# Autodesk Inventor assembly: Power Supply Board
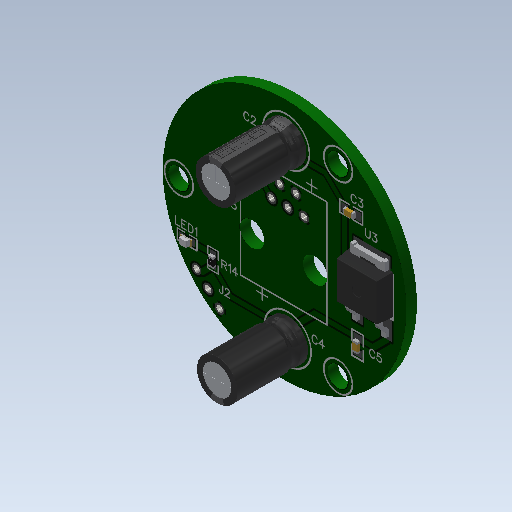
[picture p0: Inventor's stored thumbnail of the model, 512x512]
Saved by Autodesk Inventor 2020 (Build 240168000, 168)
## iProperties
Created: 2018-05-01
Part Number: Power Supply Board
Document SubType Name: Assembly
Designer: Alex
Description: 5V Regulator with RJ12 Interface
Author: Alex
## Documents named in this file (7)
- C:\Users\amsmi\Google Drive\Pirani Gauge\Pirani Gauge Modeling\Gauge Rev 3\Power Supply Board.iam
- C:\Users\amsmi\Google Drive\Pirani Gauge\Pirani Gauge Modeling\Gauge Rev 3\Power Supply.ipt
- E:\Inventor Modeling\General Parts\Electronics\Surface Mount Components\Black 0603.ipt
- E:\Inventor Modeling\General Parts\Electronics\Surface Mount Components\Cap 0603.ipt
- C:\Users\amsmi\Google Drive\Pirani Gauge\Pirani Gauge Modeling\Gauge Rev 3\aluminumelectrolytic.ipt
- E:\Inventor Modeling\General Parts\Electronics\Surface Mount Components\TO-252AA-Vishay.ipt
- C:\Users\amsmi\Google Drive\Pirani Gauge\Pirani Gauge Modeling\Gauge Rev 3\LED-0603H0.75.ipt
## Components (8 placed, 6 different names)
1. Power Supply:1 — Mate:1, Mate:2, Mate:3, Mate:4, Mate:5, Mate:6, Mate:7, Mate:8, Mate:9, Mate:10, Mate:11, Mate:12, Flush:1, Mate:14, Mate:15
2. Black 0603:1 — Mate:11, Angle:2, Flush:4, Flush:5, Flush:8, Flush:9
3. Cap 0603:1 — Mate:10, Angle:1, Angle:2, Flush:2, Flush:3, Flush:4, Flush:5, Flush:6, Flush:7
4. Cap 0603:2 — Mate:12, Mate:13, Flush:1, Angle:1, Flush:2, Flush:3
5. aluminumelectrolytic:1 — Mate:7, Mate:8, Mate:9
6. aluminumelectrolytic:2 — Mate:1, Mate:5, Mate:6
7. TO-252AA-Vishay:1 — Mate:14, Flush:6, Flush:7
8. LED-0603H0.75:1 — Mate:15, Flush:8, Flush:9
## Relationships (26: Mate 15, Flush 9, Angle 2)
- Mate:1: Power Supply:1 ↔ aluminumelectrolytic:2
- Mate:2: Power Supply:1
- Mate:3: Power Supply:1
- Mate:4: Power Supply:1
- Mate:5: Power Supply:1 ↔ aluminumelectrolytic:2
- Mate:6 (0.0508 mm): Power Supply:1 ↔ aluminumelectrolytic:2
- Mate:7: Power Supply:1 ↔ aluminumelectrolytic:1
- Mate:8: Power Supply:1 ↔ aluminumelectrolytic:1
- Mate:9 (5.2324 mm): Power Supply:1 ↔ aluminumelectrolytic:1
- Mate:10: Power Supply:1 ↔ Cap 0603:1
- Mate:11: Power Supply:1 ↔ Black 0603:1
- Mate:12: Power Supply:1 ↔ Cap 0603:2
- Mate:13 (8.4836 mm): Cap 0603:2
- Flush:1 (11.1506 mm): Power Supply:1 ↔ Cap 0603:2
- Angle:1 (90 deg): Cap 0603:1 ↔ Cap 0603:2
- Angle:2 (0 deg): Black 0603:1 ↔ Cap 0603:1
- Flush:2 (-0.7112 mm): Cap 0603:1 ↔ Cap 0603:2
- Flush:3 (-17.8816 mm): Cap 0603:1 ↔ Cap 0603:2
- Flush:4 (-22.606 mm): Black 0603:1 ↔ Cap 0603:1
- Flush:5 (0.254 mm): Black 0603:1 ↔ Cap 0603:1
- Mate:14: Power Supply:1 ↔ TO-252AA-Vishay:1
- Flush:6 (-4.5212 mm): Cap 0603:1 ↔ TO-252AA-Vishay:1
- Flush:7 (12.9794 mm): Cap 0603:1 ↔ TO-252AA-Vishay:1
- Mate:15: Power Supply:1 ↔ LED-0603H0.75:1
- Flush:8 (-4.4958 mm): Black 0603:1 ↔ LED-0603H0.75:1
- Flush:9 (0.9906 mm): Black 0603:1 ↔ LED-0603H0.75:1
